# Autodesk Inventor assembly: full battery cart
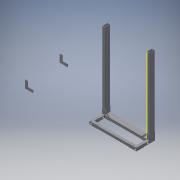
[picture p0: Inventor's stored thumbnail of the model, 180x180]
Saved by Autodesk Inventor 2018 (Build 220112000, 112)
## iProperties
Created: 2018-12-12
Part Number: full battery cart
Document SubType Name: Assembly
Designer: s-4008082
Author: s-4008082
## Documents named in this file (4)
- \\studenthome\students\S-4008082\Battery cart\full battery cart.iam
- \\studenthome\students\S-4008082\Battery cart\battery shelf frame.ipt
- \\studenthome\students\S-4008082\Battery cart\special brace.ipt
- \\studenthome\students\S-4008082\Battery cart\bracket.ipt
## Components (11 placed, 3 different names)
1. battery shelf frame:1 — Mate:1, Mate:2, Mate:3, Mate:4, Mate:5, Mate:6, Mate:7, Mate:8, Mate:9, Flush:1, Flush:2, Mate:10, Flush:3, Flush:4, Mate:11, Flush:5, Mate:12, Mate:13, Mate:14, Mate:15, Mate:16, Mate:17, Mate:18, Mate:19
2. special brace:1 — Mate:6, Mate:7, Mate:8
3. special brace:2 — Mate:3, Mate:4, Mate:5
4. bracket:1 — Mate:1, Mate:2
5. bracket:2 — Mate:11, Flush:5, Mate:12
6. bracket:3
7. bracket:4 — Mate:17, Mate:18, Mate:19
8. bracket:5 — Mate:10, Flush:3, Flush:4
9. bracket:6
10. bracket:7 — Mate:13, Mate:14, Mate:15, Mate:16
11. bracket:8 — Mate:9, Flush:1, Flush:2
## Relationships (24: Mate 19, Flush 5)
- Mate:1: battery shelf frame:1 ↔ bracket:1
- Mate:2: battery shelf frame:1 ↔ bracket:1
- Mate:3: battery shelf frame:1 ↔ special brace:2
- Mate:4: battery shelf frame:1 ↔ special brace:2
- Mate:5: battery shelf frame:1 ↔ special brace:2
- Mate:6: battery shelf frame:1 ↔ special brace:1
- Mate:7: battery shelf frame:1 ↔ special brace:1
- Mate:8: battery shelf frame:1 ↔ special brace:1
- Mate:9: battery shelf frame:1 ↔ bracket:8
- Flush:1: battery shelf frame:1 ↔ bracket:8
- Flush:2: battery shelf frame:1 ↔ bracket:8
- Mate:10: battery shelf frame:1 ↔ bracket:5
- Flush:3: battery shelf frame:1 ↔ bracket:5
- Flush:4: battery shelf frame:1 ↔ bracket:5
- Mate:11: battery shelf frame:1 ↔ bracket:2
- Flush:5: battery shelf frame:1 ↔ bracket:2
- Mate:12: battery shelf frame:1 ↔ bracket:2
- Mate:13: battery shelf frame:1 ↔ bracket:7
- Mate:14: battery shelf frame:1 ↔ bracket:7
- Mate:15: battery shelf frame:1 ↔ bracket:7
- Mate:16: battery shelf frame:1 ↔ bracket:7
- Mate:17: battery shelf frame:1 ↔ bracket:4
- Mate:18: battery shelf frame:1 ↔ bracket:4
- Mate:19: battery shelf frame:1 ↔ bracket:4
